# Autodesk Inventor assembly: dsitributor
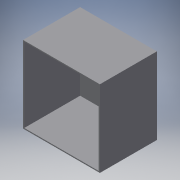
[picture p0: Inventor's stored thumbnail of the model, 180x180]
Saved by Autodesk Inventor 2018 (Build 220112000, 112)
## iProperties
Created: 2018-12-03
Part Number: dsitributor
Document SubType Name: Assembly
Designer: Bienvenue
Author: Bienvenue
## Documents named in this file (4)
- C:\Users\Bienvenue\Documents\Cours\PeiP2\Arduino\Projet\Monnayeur\dsitributor.iam
- C:\Users\Bienvenue\Documents\Cours\PeiP2\Arduino\Projet\Monnayeur\planche_gauche.ipt
- C:\Users\Bienvenue\Documents\Cours\PeiP2\Arduino\Projet\Monnayeur\planche derrière.ipt
- C:\Users\Bienvenue\Documents\Cours\PeiP2\Arduino\Projet\planche_bas.ipt
## Components (5 placed, 3 different names)
1. planche_gauche:1 — Mate:1, Flush:1, Flush:3, Flush:6, Mate:4, Mate:5
2. planche_gauche:2 — Mate:2, Flush:2, Flush:4, Flush:5, Flush:8
3. planche derrière:1 — Mate:3, Flush:5, Flush:6, Mate:4, Flush:7
4. planche_bas:1 — Mate:1, Mate:2, Flush:1, Flush:2, Flush:3, Flush:4, Mate:3
5. planche_bas:2 — Mate:5, Flush:7, Flush:8
## Relationships (13: Flush 8, Mate 5)
- Mate:1: planche_gauche:1 ↔ planche_bas:1
- Mate:2: planche_gauche:2 ↔ planche_bas:1
- Flush:1: planche_gauche:1 ↔ planche_bas:1
- Flush:2: planche_gauche:2 ↔ planche_bas:1
- Flush:3: planche_gauche:1 ↔ planche_bas:1
- Flush:4: planche_gauche:2 ↔ planche_bas:1
- Mate:3: planche derrière:1 ↔ planche_bas:1
- Flush:5: planche_gauche:2 ↔ planche derrière:1
- Flush:6: planche_gauche:1 ↔ planche derrière:1
- Mate:4: planche_gauche:1 ↔ planche derrière:1
- Mate:5: planche_gauche:1 ↔ planche_bas:2
- Flush:7: planche derrière:1 ↔ planche_bas:2
- Flush:8: planche_gauche:2 ↔ planche_bas:2
